# Autodesk Inventor assembly: powersupply assm
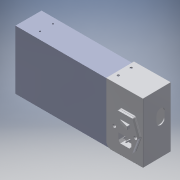
[picture p0: Inventor's stored thumbnail of the model, 180x180]
Saved by Autodesk Inventor 2017 (Build 210142000, 142)
## iProperties
Created: 2018-07-05
Part Number: powersupply assm
Document SubType Name: Assembly
Designer: UnKnoWn
Author: UnKnoWn
## Documents named in this file (4)
- I:\3d Printer stuff\Ender 3\Ender3 working files\Ender-3 Mechanical\STP\powersupply assm.iam
- I:\3d Printer stuff\Ender 3\Ender3 working files\Ender-3 Mechanical\STP\24V15A power supply.ipt
- I:\3d Printer stuff\Ender 3\Ender3 working files\Ender-3 Mechanical\STP\Power holder.ipt
- I:\3d Printer stuff\Ender 3\Ender3 working files\Ender-3 Mechanical\STP\power switch.ipt
## Components (3 placed, 3 different names)
1. 24V15A power supply:1 — Mate:1, Mate:2
2. Power holder:1 — Mate:1, Mate:2, Mate:3, Mate:4
3. power switch:1 — Mate:3, Mate:4
## Relationships (4: Mate 4)
- Mate:1: 24V15A power supply:1 ↔ Power holder:1
- Mate:2: 24V15A power supply:1 ↔ Power holder:1
- Mate:3: Power holder:1 ↔ power switch:1
- Mate:4: Power holder:1 ↔ power switch:1
